# Autodesk Inventor assembly: 针头主体
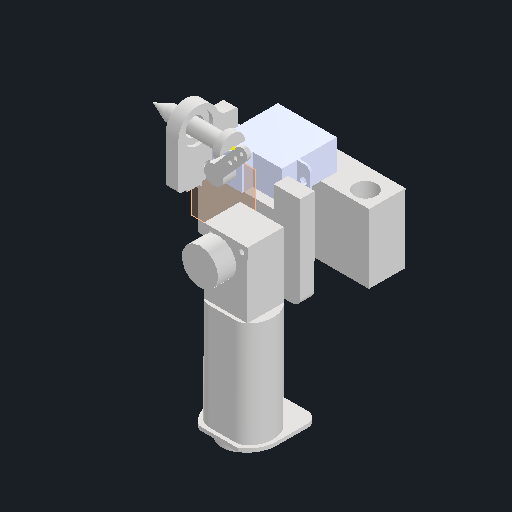
[picture p0: Inventor's stored thumbnail of the model, 512x512]
Saved by Autodesk Inventor 2025 (Build 290162000, 162)
## iProperties
Created: 2025-12-02
Part Number: 针头主体
Document SubType Name: Assembly
Designer: XH
Author: XH
## Documents named in this file (9)
- D:\2 B Mechanical design\braille-printer-v2\针头主体.iam
- D:\2 B Mechanical design\braille-printer-v2\小舵机.ipt
- D:\2 B Mechanical design\braille-printer-v2\针头.ipt
- D:\2 B Mechanical design\braille-printer-v2\摆臂.ipt
- D:\2 B Mechanical design\braille-printer-v2\针头装配体.ipt
- D:\2 B Mechanical design\braille-printer-v2\电机.ipt
- D:\2 B Mechanical design\braille-printer-v2\电机装配.ipt
- D:\2 B Mechanical design\braille-printer-v2\皮带轮.ipt
- D:\2 B Mechanical design\braille-printer-v2\固定传动.ipt
## Components (8 placed, 8 different names)
1. 小舵机:1 — 配合:1, 配合:2, 配合:4
2. 针头:1 — 配合:3
3. 摆臂:1 — 配合:1, 配合:2
4. 针头装配体:1 — 配合:3, 配合:4, 配合:8, 配合:9, 配合:11
5. 电机:1 — 配合:10, 配合:12, 配合:14, 配合:15
6. 电机装配:1 — 配合:8, 配合:9, 配合:10, 配合:11, 配合:12, 配合:15, 配合:16, 表面齐平:1, 表面齐平:2
7. 皮带轮:1 — 配合:14
8. 固定传动:1 — 配合:16, 表面齐平:1, 表面齐平:2
## Relationships (14: Mate 12, Flush 2)
- 配合:1 [Mate]: 小舵机:1 ↔ 摆臂:1
- 配合:2 [Mate]: 小舵机:1 ↔ 摆臂:1
- 配合:3 [Mate]: 针头:1 ↔ 针头装配体:1
- 配合:4 [Mate]: 小舵机:1 ↔ 针头装配体:1
- 配合:8 [Mate]: 针头装配体:1 ↔ 电机装配:1
- 配合:9 [Mate]: 针头装配体:1 ↔ 电机装配:1
- 配合:10 [Mate]: 电机:1 ↔ 电机装配:1
- 配合:11 [Mate]: 针头装配体:1 ↔ 电机装配:1
- 配合:12 [Mate]: 电机:1 ↔ 电机装配:1
- 配合:14 [Mate]: 电机:1 ↔ 皮带轮:1
- 配合:15 [Mate]: 电机:1 ↔ 电机装配:1
- 配合:16 [Mate]: 电机装配:1 ↔ 固定传动:1
- 表面齐平:1 [Flush]: 电机装配:1 ↔ 固定传动:1
- 表面齐平:2 [Flush]: 电机装配:1 ↔ 固定传动:1
